# Autodesk Inventor assembly: Full payload assembly mk 2
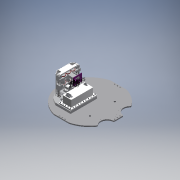
[picture p0: Inventor's stored thumbnail of the model, 180x180]
Saved by Autodesk Inventor 2017 (Build 210142000, 142)
## iProperties
Created: 2016-12-06
Part Number: Full payload assembly mk 2
Document SubType Name: Assembly
Designer: qupec
Mass: 1513.48 g
Surface Area: 2866.97 cm^2
Volume: 582.995 cm^3
Density: 2.59604 g/cm^3
Author: qupec
## Documents named in this file (42)
- C:\UMD\BPP\ROCKSAT X\STAR\CAD\Mechanical\Full payload assembly\Full payload assembly.iam
- C:\UMD\BPP\ROCKSAT X\STAR\CAD\Mechanical\Full payload assembly\Subsystems\Slide Rods\Slide rod assembly.iam
- C:\UMD\BPP\ROCKSAT X\STAR\CAD\Mechanical\Full payload assembly\Subsystems\Test Tube Rack\Test tube rack.iam
- C:\UMD\BPP\ROCKSAT X\STAR\CAD\Mechanical\Full payload assembly\Subsystems\Electronics\Electronics Stack.iam
- C:\UMD\BPP\ROCKSAT X\STAR\CAD\Mechanical\Full payload assembly\Subsystems\Video Capture\Pi Cam and Cable assembly.iam
- C:\UMD\BPP\ROCKSAT X\STAR\CAD\Mechanical\Full payload assembly\Subsystems\Electronics\Ribbon Cable Connector-02.ipt
- C:\UMD\BPP\ROCKSAT X\STAR\CAD\Mechanical\Full payload assembly\Base Plate.ipt
- C:\UMD\BPP\ROCKSAT X\STAR\CAD\Mechanical\Full payload assembly\Subsystems\Electronics\Electronics Box.ipt
- C:\UMD\BPP\ROCKSAT X\STAR\CAD\Mechanical\Full payload assembly\Subsystems\Electronics\External Sensor Board.ipt
- C:\UMD\BPP\ROCKSAT X\STAR\CAD\Mechanical\Full payload assembly\Subsystems\Electronics\9pin female connector.ipt
- C:\UMD\BPP\ROCKSAT X\STAR\CAD\Mechanical\Full payload assembly\Subsystems\Electronics\31pin female connector.ipt
- C:\UMD\BPP\ROCKSAT X\STAR\CAD\Mechanical\Full payload assembly\Subsystems\Electronics\15pin female connector.ipt
- C:\UMD\BPP\ROCKSAT X\STAR\CAD\Mechanical\Full payload assembly\Subsystems\Video Capture\LED.ipt
- C:\UMD\BPP\ROCKSAT X\STAR\CAD\Mechanical\Full payload assembly\Solar Shield.ipt
- C:\UMD\BPP\ROCKSAT X\STAR\CAD\Mechanical\Full payload assembly\BRACKET.ipt
- C:\UMD\BPP\ROCKSAT X\STAR\CAD\Mechanical\Full payload assembly\Subsystems\Shaker\ShakerAssembly.iam
- C:\UMD\BPP\ROCKSAT X\STAR\CAD\Mechanical\Full payload assembly\Subsystems\Fasteners\Num4 Narrow Split Washer.ipt
- C:\UMD\BPP\ROCKSAT X\STAR\CAD\Mechanical\Full payload assembly\Subsystems\Fasteners\4-40 .5in Socket Screw.ipt
- C:\UMD\BPP\ROCKSAT X\STAR\CAD\Mechanical\Full payload assembly\Subsystems\Fasteners\4-40 .375in Countersunk Screw.ipt
- C:\UMD\BPP\ROCKSAT X\STAR\CAD\Mechanical\Full payload assembly\Subsystems\Fasteners\Num4 Flat Washer.ipt
- C:\UMD\BPP\ROCKSAT X\STAR\CAD\Mechanical\Full payload assembly\Subsystems\Fasteners\4-40 Flex Nut.ipt
- C:\UMD\BPP\ROCKSAT X\STAR\CAD\Mechanical\Full payload assembly\Subsystems\Fasteners\4-40 .375 Socket Screw.ipt
- C:\UMD\BPP\ROCKSAT X\STAR\CAD\Mechanical\Full payload assembly\RSX Deck.ipt
- C:\UMD\BPP\ROCKSAT X\STAR\CAD\Mechanical\Full payload assembly\Subsystems\Fasteners\Num10 Belville Washer.ipt
- C:\UMD\BPP\ROCKSAT X\STAR\CAD\Mechanical\Full payload assembly\Subsystems\Fasteners\10-32 .375in Low Profile Socket Screw.ipt
- C:\UMD\BPP\ROCKSAT X\STAR\CAD\Mechanical\Full payload assembly\Subsystems\Fasteners\10-32 1.125in Countersunk Screw.ipt
- C:\UMD\BPP\ROCKSAT X\STAR\CAD\Mechanical\Full payload assembly\Subsystems\Fasteners\10-32 Flex Nut.ipt
- C:\UMD\BPP\ROCKSAT X\STAR\CAD\Mechanical\Full payload assembly\Subsystems\Fasteners\M2 Insulating Washer.ipt
- C:\UMD\BPP\ROCKSAT X\STAR\CAD\Mechanical\Full payload assembly\Subsystems\Fasteners\M2x.4mm Locknut.ipt
- C:\UMD\BPP\ROCKSAT X\STAR\CAD\Mechanical\Full payload assembly\Subsystems\Fasteners\M2x.4mm 12mm Socket Screw.ipt
- C:\UMD\BPP\ROCKSAT X\star\CAD\Mechanical\Subsystems\Full payload assembly mk 2\AIP\FEA\c3occb59c.fins
- C:\UMD\BPP\ROCKSAT X\star\CAD\Mechanical\Subsystems\Full payload assembly mk 2\AIP\FEA\c3occb5b4.fsat
- C:\UMD\BPP\ROCKSAT X\star\CAD\Mechanical\Subsystems\Full payload assembly mk 2\AIP\FEA\c3occb5b4.ftes
- C:\UMD\BPP\ROCKSAT X\star\CAD\Mechanical\Subsystems\Full payload assembly mk 2\AIP\FEA\c3occb5b4.fwiz
- C:\UMD\BPP\ROCKSAT X\star\CAD\Mechanical\Subsystems\Full payload assembly mk 2\AIP\FEA\c3occb5c0.fins
- C:\UMD\BPP\ROCKSAT X\star\CAD\Mechanical\Subsystems\Full payload assembly mk 2\AIP\FEA\c3occb5c0.fsat
- C:\UMD\BPP\ROCKSAT X\star\CAD\Mechanical\Subsystems\Full payload assembly mk 2\AIP\FEA\c3occb5c0.ftes
- C:\UMD\BPP\ROCKSAT X\star\CAD\Mechanical\Subsystems\Full payload assembly mk 2\AIP\FEA\c3occb5c0.fwiz
- C:\UMD\BPP\ROCKSAT X\star\CAD\Mechanical\Subsystems\Full payload assembly mk 2\AIP\FEA\c3occb60w.fmsh
- C:\UMD\BPP\ROCKSAT X\star\CAD\Mechanical\Subsystems\Full payload assembly mk 2\AIP\FEA\c3occb60x.fres
- C:\UMD\BPP\ROCKSAT X\star\CAD\Mechanical\Subsystems\Full payload assembly mk 2\AIP\FEA\c3occb6sg.fmsh
- C:\UMD\BPP\ROCKSAT X\star\CAD\Mechanical\Subsystems\Full payload assembly mk 2\AIP\FEA\c3occb6sh.fres
## Components (134 placed, 29 different names)
1. Slide rod assembly:1 [sub-assembly] — Mate:121, Flush:47, Mate:382, Mate:398, Mate:399, Flush:48
2. Test tube rack:1 [sub-assembly] — Mate:56, Flush:19, Flush:20, Flush:45, Mate:395, Mate:396, Mate:398, Mate:399, Mate:629, Mate:632, Mate:633, Mate:637, Mate:638
3. Pi Cam and Cable assembly:1 [sub-assembly] — Mate:56, Flush:19, Flush:20, Mate:299, Mate:300, Mate:302, Mate:303, Mate:304, Mate:593, Mate:594, Mate:595, Mate:596, Mate:597, Mate:598, Mate:599, Mate:600, Mate:606, Mate:625, Mate:626, Mate:627, Mate:628, Mate:630, Mate:631, Mate:636
4. Ribbon Cable Connector-02:1 — Mate:80, Flush:24, Flush:25
5. Electronics Stack:1 [sub-assembly] — Mate:80, Flush:24, Flush:25, Flush:41, Flush:42, Mate:397
6. Base Plate:1 — Mate:121, Mate:124, Flush:29, Flush:32, Mate:163, Flush:33, Flush:40, Flush:45, Mate:386, Mate:389, Mate:392, Mate:393, Mate:394, Mate:397, Mate:559, Mate:560, Mate:561, Mate:589, Mate:590, Mate:591, Mate:592
7. External Sensor Board:1 — Angle:1, Mate:303, Mate:304, Mate:305, Mate:306, Mate:609, Mate:610, Mate:611, Mate:612, Mate:613, Mate:614, Mate:615, Mate:616
8. 31pin female connector:1 — Flush:34, Flush:35, Mate:164
9. 15pin female connector:1 — Mate:165, Flush:43, Flush:44
10. 9pin female connector:1 — Flush:38, Flush:39, Mate:166
11. Electronics Box:1 — Mate:163, Flush:33, Flush:34, Flush:35, Mate:164, Flush:38, Flush:39, Mate:165, Mate:166, Flush:40, Flush:41, Flush:42, Flush:43, Flush:44, Mate:400, Mate:401, Mate:402, Mate:403, Mate:404, Mate:405, Mate:406, Mate:407, Mate:408, Mate:409, Mate:410, Mate:411, Mate:412, Mate:413, Mate:414, Mate:415, Mate:416, Mate:417, Mate:418, Mate:419, Mate:420, Mate:421, Mate:422, Mate:423, Mate:424, Mate:425, Mate:426, Mate:427, Mate:428, Mate:429, Mate:430, Mate:431, Mate:432, Mate:433, Mate:434, Mate:435, Mate:437, Mate:438, Mate:439, Mate:440, Mate:441, Mate:442, Mate:443, Mate:444, Mate:445, Mate:446, Mate:447, Mate:448, Mate:449, Mate:450, Mate:451, Mate:452, Mate:453, Mate:454, Mate:455, Mate:456, Mate:457, Mate:458, Mate:459, Mate:518
12. LED:1 — Mate:299, Mate:301, Mate:302, Mate:305
13. LED:2 — Mate:300, Mate:301, Mate:306
14. Solar Shield:1 — Flush:47, Mate:382, Mate:387, Mate:388, Mate:390, Mate:391, Mate:536, Mate:538, Mate:540, Mate:542, Mate:551, Mate:552, Mate:553, Mate:554, Mate:557, Mate:558, Flush:48
15. BRACKET:1 — Mate:389, Mate:390, Mate:391, Mate:519, Mate:520, Mate:521, Mate:522, Mate:527, Mate:528, Mate:529, Mate:530
16. BRACKET:2 — Mate:386, Mate:387, Mate:388, Mate:523, Mate:524, Mate:525, Mate:526, Mate:531, Mate:532, Mate:533, Mate:534
17. ShakerAssembly:1 [sub-assembly] — Mate:392, Mate:393, Mate:394, Mate:395, Mate:396
18. Num4 Narrow Split Washer:1 — Mate:411, Mate:457, Mate:645
19. Num4 Narrow Split Washer:2 — Mate:413, Mate:419, Mate:455
20. Num4 Narrow Split Washer:3 — Mate:415, Mate:450
21. Num4 Narrow Split Washer:4 — Mate:414, Mate:444
22. Num4 Narrow Split Washer:5 — Mate:412, Mate:452
23. Num4 Narrow Split Washer:6 — Mate:410, Mate:443
24. Num4 Narrow Split Washer:7 — Mate:409, Mate:453
25. Num4 Narrow Split Washer:8 — Mate:408, Mate:441
26. Num4 Narrow Split Washer:9 — Mate:420, Mate:437
27. Num4 Narrow Split Washer:10 — Mate:423, Mate:451
28. Num4 Narrow Split Washer:11 — Mate:407, Mate:445
29. Num4 Narrow Split Washer:12 — Mate:405, Mate:447
30. Num4 Narrow Split Washer:13 — Mate:428, Mate:433
31. Num4 Narrow Split Washer:14 — Mate:426, Mate:435
32. Num4 Narrow Split Washer:15 — Mate:418, Mate:430
33. Num4 Narrow Split Washer:17 — Mate:422, Mate:454
34. Num4 Narrow Split Washer:18 — Mate:417, Mate:431
35. Num4 Narrow Split Washer:19 — Mate:425, Mate:456
36. Num4 Narrow Split Washer:20 — Mate:424, Mate:439
37. Num4 Narrow Split Washer:21 — Mate:427, Mate:434
38. Num4 Narrow Split Washer:22 — Mate:429, Mate:432
39. Num4 Narrow Split Washer:23 — Mate:421, Mate:438
40. Num4 Narrow Split Washer:24 — Mate:404, Mate:440
41. Num4 Narrow Split Washer:25 — Mate:401, Mate:442
42. Num4 Narrow Split Washer:26 — Mate:400, Mate:416, Mate:449
43. Num4 Narrow Split Washer:27 — Mate:402, Mate:406, Mate:446
44. Num4 Narrow Split Washer:28 — Mate:403, Mate:448
45. Num4 Narrow Split Washer:29 — Mate:458, Mate:459
46. 4-40 .5in Socket Screw:1
47. 4-40 .5in Socket Screw:2
48. 4-40 .5in Socket Screw:3
49. 4-40 .5in Socket Screw:4
50. 4-40 .5in Socket Screw:5
51. 4-40 .5in Socket Screw:6
52. 4-40 .5in Socket Screw:7
53. 4-40 .5in Socket Screw:8
54. 4-40 .5in Socket Screw:9
55. 4-40 .5in Socket Screw:10
56. 4-40 .5in Socket Screw:11
57. 4-40 .5in Socket Screw:12
58. 4-40 .5in Socket Screw:13
59. 4-40 .5in Socket Screw:14
60. 4-40 .5in Socket Screw:15 — Mate:518
61. 4-40 .5in Socket Screw:16
62. 4-40 .5in Socket Screw:17 — Mate:645
63. 4-40 .5in Socket Screw:18
64. 4-40 .5in Socket Screw:19
65. 4-40 .5in Socket Screw:20
66. 4-40 .5in Socket Screw:21
67. 4-40 .5in Socket Screw:22
68. 4-40 .5in Socket Screw:23
69. 4-40 .5in Socket Screw:24
70. 4-40 .5in Socket Screw:25
71. 4-40 .5in Socket Screw:26
72. 4-40 .5in Socket Screw:27
73. 4-40 .5in Socket Screw:28
74. 4-40 .375in Countersunk Screw:1 — Mate:520, Mate:521
75. 4-40 .375in Countersunk Screw:2 — Mate:519, Mate:522
76. 4-40 .375in Countersunk Screw:3 — Mate:523, Mate:526
77. 4-40 .375in Countersunk Screw:4 — Mate:524, Mate:525
78. 4-40 .375in Countersunk Screw:5 — Mate:531, Mate:534, Mate:537, Mate:546
79. 4-40 .375in Countersunk Screw:6 — Mate:528, Mate:529, Mate:541, Mate:550
80. 4-40 .375in Countersunk Screw:7 — Mate:532, Mate:533, Mate:535, Mate:543
81. 4-40 .375in Countersunk Screw:8 — Mate:527, Mate:530, Mate:539, Mate:548
82. Num4 Flat Washer:1 — Mate:539, Mate:540, Mate:547
83. Num4 Flat Washer:2 — Mate:537, Mate:538, Mate:545
84. Num4 Flat Washer:3 — Mate:535, Mate:536, Mate:544
85. Num4 Flat Washer:4 — Mate:541, Mate:542, Mate:549
86. 4-40 Flex Nut:1 — Mate:549, Mate:550
87. 4-40 Flex Nut:2 — Mate:545, Mate:546
88. 4-40 Flex Nut:3 — Mate:547, Mate:548
89. 4-40 Flex Nut:4 — Mate:543, Mate:544
90. Num4 Narrow Split Washer:30 — Mate:551, Mate:552, Mate:556
91. Num4 Narrow Split Washer:31 — Mate:553, Mate:554, Mate:555
92. 4-40 .375 Socket Screw:1 — Mate:555, Mate:558
93. 4-40 .375 Socket Screw:2 — Mate:556, Mate:557
94. RSX Deck:1 — Mate:559, Mate:560, Mate:561, Mate:562, Mate:563, Mate:565, Mate:566, Mate:567, Mate:568, Mate:569, Mate:570, Mate:571, Mate:575, Mate:577, Mate:578, Mate:579, Mate:580, Mate:581, Mate:582, Mate:583, Mate:584
95. Num10 Belville Washer:1 — Mate:562, Mate:563, Mate:574
96. Num10 Belville Washer:3 — Mate:565, Mate:566, Mate:573
97. Num10 Belville Washer:4 — Mate:567, Mate:568, Mate:572
98. 10-32 .375in Low Profile Socket Screw:1 — Mate:569, Mate:574
99. 10-32 .375in Low Profile Socket Screw:2 — Mate:570, Mate:573
100. 10-32 .375in Low Profile Socket Screw:3 — Mate:571, Mate:572
101. 10-32 1.125in Countersunk Screw:1 — Mate:575, Mate:581, Mate:582, Mate:585
102. 10-32 1.125in Countersunk Screw:2 — Mate:577, Mate:584, Mate:587
103. 10-32 1.125in Countersunk Screw:3 — Mate:579, Mate:580, Mate:586
104. 10-32 1.125in Countersunk Screw:4 — Mate:578, Mate:583, Mate:588
105. 10-32 Flex Nut:1 — Mate:586, Mate:589
106. 10-32 Flex Nut:2 — Mate:587, Mate:592
107. 10-32 Flex Nut:3 — Mate:588, Mate:591
108. 10-32 Flex Nut:4 — Mate:585, Mate:590
109. M2 Insulating Washer:1 — Mate:593, Mate:594, Mate:603, Mate:604
110. M2 Insulating Washer:2 — Mate:599, Mate:600, Mate:607, Mate:608
111. M2 Insulating Washer:3 — Mate:597, Mate:598, Mate:605
112. M2 Insulating Washer:4 — Mate:595, Mate:596, Mate:601, Mate:602
113. M2x.4mm Locknut:1 — Mate:601, Mate:602
114. M2x.4mm Locknut:2 — Mate:603, Mate:604
115. M2x.4mm Locknut:3 — Mate:607, Mate:608
116. M2x.4mm Locknut:4 — Mate:605, Mate:606
117. M2x.4mm 12mm Socket Screw:1 — Mate:610, Mate:619, Mate:623
118. M2x.4mm 12mm Socket Screw:2 — Mate:609, Mate:618, Mate:621
119. M2x.4mm 12mm Socket Screw:3 — Mate:611, Mate:617, Mate:622
120. M2x.4mm 12mm Socket Screw:4 — Mate:612, Mate:620, Mate:624
121. M2 Insulating Washer:5 — Mate:616, Mate:617
122. M2 Insulating Washer:6 — Mate:614, Mate:619
123. M2 Insulating Washer:7 — Mate:613, Mate:620, Mate:624
124. M2 Insulating Washer:8 — Mate:615, Mate:618, Mate:621, Mate:622, Mate:623
125. Num4 Flat Washer:5 — Mate:625, Mate:630, Mate:634, Mate:635
126. Num4 Flat Washer:6 — Mate:627, Mate:629
127. Num4 Flat Washer:7 — Mate:626, Mate:628
128. 4-40 .5in Socket Screw:29 — Mate:631, Mate:636, Mate:639, Mate:644
129. 4-40 .5in Socket Screw:30 — Mate:632, Mate:634, Mate:640, Mate:643
130. 4-40 .5in Socket Screw:31 — Mate:633, Mate:635
131. Num4 Flat Washer:8 — Mate:637, Mate:640, Mate:642
132. Num4 Flat Washer:9 — Mate:638, Mate:639, Mate:641
133. 4-40 Flex Nut:5 — Mate:642, Mate:643
134. 4-40 Flex Nut:6 — Mate:641, Mate:644
## Relationships (291: Mate 271, Flush 19, Angle 1)
- Mate:56: Test tube rack:1 ↔ Pi Cam and Cable assembly:1
- Flush:19: Test tube rack:1 ↔ Pi Cam and Cable assembly:1
- Flush:20: Test tube rack:1 ↔ Pi Cam and Cable assembly:1
- Mate:80: Ribbon Cable Connector-02:1 ↔ Electronics Stack:1
- Flush:24 (-7 mm): Ribbon Cable Connector-02:1 ↔ Electronics Stack:1
- Flush:25: Ribbon Cable Connector-02:1 ↔ Electronics Stack:1
- Mate:121: Slide rod assembly:1 ↔ Base Plate:1
- Mate:124: Base Plate:1
- Flush:29: Base Plate:1
- Flush:32: Base Plate:1
- Angle:1 (0 deg): External Sensor Board:1
- Mate:163: Base Plate:1 ↔ Electronics Box:1
- Flush:33: Base Plate:1 ↔ Electronics Box:1
- Flush:34 (12.7 mm): 31pin female connector:1 ↔ Electronics Box:1
- Flush:35 (6.35 mm): 31pin female connector:1 ↔ Electronics Box:1
- Mate:164: 31pin female connector:1 ↔ Electronics Box:1
- Flush:38 (6.35 mm): 9pin female connector:1 ↔ Electronics Box:1
- Flush:39 (-6.35 mm): 9pin female connector:1 ↔ Electronics Box:1
- Mate:165: 15pin female connector:1 ↔ Electronics Box:1
- Mate:166: 9pin female connector:1 ↔ Electronics Box:1
- Flush:40: Base Plate:1 ↔ Electronics Box:1
- Flush:41 (3.175 mm): Electronics Stack:1 ↔ Electronics Box:1
- Flush:42: Electronics Stack:1 ↔ Electronics Box:1
- Flush:43 (3.81 mm): 15pin female connector:1 ↔ Electronics Box:1
- Flush:44 (12.7 mm): 15pin female connector:1 ↔ Electronics Box:1
- Mate:299: Pi Cam and Cable assembly:1 ↔ LED:1
- Mate:300: Pi Cam and Cable assembly:1 ↔ LED:2
- Mate:301: LED:1 ↔ LED:2
- Mate:302: Pi Cam and Cable assembly:1 ↔ LED:1
- Mate:303: Pi Cam and Cable assembly:1 ↔ External Sensor Board:1
- Mate:304: Pi Cam and Cable assembly:1 ↔ External Sensor Board:1
- Mate:305: External Sensor Board:1 ↔ LED:1
- Mate:306: External Sensor Board:1 ↔ LED:2
- Flush:45: Test tube rack:1 ↔ Base Plate:1
- Flush:47: Slide rod assembly:1 ↔ Solar Shield:1
- Mate:382: Slide rod assembly:1 ↔ Solar Shield:1
- Mate:386: Base Plate:1 ↔ BRACKET:2
- Mate:387: Solar Shield:1 ↔ BRACKET:2
- Mate:388 (3.175 mm): Solar Shield:1 ↔ BRACKET:2
- Mate:389: Base Plate:1 ↔ BRACKET:1
- Mate:390: Solar Shield:1 ↔ BRACKET:1
- Mate:391 (3.175 mm): Solar Shield:1 ↔ BRACKET:1
- Mate:392: Base Plate:1 ↔ ShakerAssembly:1
- Mate:393: Base Plate:1 ↔ ShakerAssembly:1
- Mate:394: Base Plate:1 ↔ ShakerAssembly:1
- Mate:395: Test tube rack:1 ↔ ShakerAssembly:1
- Mate:396: Test tube rack:1 ↔ ShakerAssembly:1
- Mate:397: Electronics Stack:1 ↔ Base Plate:1
- Mate:398: Slide rod assembly:1 ↔ Test tube rack:1
- Mate:399: Slide rod assembly:1 ↔ Test tube rack:1
- Mate:400: Electronics Box:1 ↔ Num4 Narrow Split Washer:26
- Mate:401: Electronics Box:1 ↔ Num4 Narrow Split Washer:25
- Mate:402: Electronics Box:1 ↔ Num4 Narrow Split Washer:27
- Mate:403: Electronics Box:1 ↔ Num4 Narrow Split Washer:28
- Mate:404: Electronics Box:1 ↔ Num4 Narrow Split Washer:24
- Mate:405: Electronics Box:1 ↔ Num4 Narrow Split Washer:12
- Mate:406: Electronics Box:1 ↔ Num4 Narrow Split Washer:27
- Mate:407: Electronics Box:1 ↔ Num4 Narrow Split Washer:11
- Mate:408: Electronics Box:1 ↔ Num4 Narrow Split Washer:8
- Mate:409: Electronics Box:1 ↔ Num4 Narrow Split Washer:7
- Mate:410: Electronics Box:1 ↔ Num4 Narrow Split Washer:6
- Mate:411: Electronics Box:1 ↔ Num4 Narrow Split Washer:1
- Mate:412: Electronics Box:1 ↔ Num4 Narrow Split Washer:5
- Mate:413: Electronics Box:1 ↔ Num4 Narrow Split Washer:2
- Mate:414: Electronics Box:1 ↔ Num4 Narrow Split Washer:4
- Mate:415: Electronics Box:1 ↔ Num4 Narrow Split Washer:3
- Mate:416: Electronics Box:1 ↔ Num4 Narrow Split Washer:26
- Mate:417: Electronics Box:1 ↔ Num4 Narrow Split Washer:18
- Mate:418: Electronics Box:1 ↔ Num4 Narrow Split Washer:15
- Mate:419: Electronics Box:1 ↔ Num4 Narrow Split Washer:2
- Mate:420: Electronics Box:1 ↔ Num4 Narrow Split Washer:9
- Mate:421: Electronics Box:1 ↔ Num4 Narrow Split Washer:23
- Mate:422: Electronics Box:1 ↔ Num4 Narrow Split Washer:17
- Mate:423: Electronics Box:1 ↔ Num4 Narrow Split Washer:10
- Mate:424: Electronics Box:1 ↔ Num4 Narrow Split Washer:20
- Mate:425: Electronics Box:1 ↔ Num4 Narrow Split Washer:19
- Mate:426: Electronics Box:1 ↔ Num4 Narrow Split Washer:14
- Mate:427: Electronics Box:1 ↔ Num4 Narrow Split Washer:21
- Mate:428: Electronics Box:1 ↔ Num4 Narrow Split Washer:13
- Mate:429: Electronics Box:1 ↔ Num4 Narrow Split Washer:22
- Mate:430: Electronics Box:1 ↔ Num4 Narrow Split Washer:15
- Mate:431: Electronics Box:1 ↔ Num4 Narrow Split Washer:18
- Mate:432: Electronics Box:1 ↔ Num4 Narrow Split Washer:22
- Mate:433: Electronics Box:1 ↔ Num4 Narrow Split Washer:13
- Mate:434: Electronics Box:1 ↔ Num4 Narrow Split Washer:21
- Mate:435: Electronics Box:1 ↔ Num4 Narrow Split Washer:14
- Mate:437: Electronics Box:1 ↔ Num4 Narrow Split Washer:9
- Mate:438: Electronics Box:1 ↔ Num4 Narrow Split Washer:23
- Mate:439: Electronics Box:1 ↔ Num4 Narrow Split Washer:20
- Mate:440: Electronics Box:1 ↔ Num4 Narrow Split Washer:24
- Mate:441: Electronics Box:1 ↔ Num4 Narrow Split Washer:8
- Mate:442: Electronics Box:1 ↔ Num4 Narrow Split Washer:25
- Mate:443: Electronics Box:1 ↔ Num4 Narrow Split Washer:6
- Mate:444: Electronics Box:1 ↔ Num4 Narrow Split Washer:4
- Mate:445: Electronics Box:1 ↔ Num4 Narrow Split Washer:11
- Mate:446: Electronics Box:1 ↔ Num4 Narrow Split Washer:27
- Mate:447: Electronics Box:1 ↔ Num4 Narrow Split Washer:12
- Mate:448: Electronics Box:1 ↔ Num4 Narrow Split Washer:28
- Mate:449: Electronics Box:1 ↔ Num4 Narrow Split Washer:26
- Mate:450: Electronics Box:1 ↔ Num4 Narrow Split Washer:3
- Mate:451: Electronics Box:1 ↔ Num4 Narrow Split Washer:10
- Mate:452: Electronics Box:1 ↔ Num4 Narrow Split Washer:5
- Mate:453: Electronics Box:1 ↔ Num4 Narrow Split Washer:7
- Mate:454: Electronics Box:1 ↔ Num4 Narrow Split Washer:17
- Mate:455: Electronics Box:1 ↔ Num4 Narrow Split Washer:2
- Mate:456: Electronics Box:1 ↔ Num4 Narrow Split Washer:19
- Mate:457: Electronics Box:1 ↔ Num4 Narrow Split Washer:1
- Mate:458: Electronics Box:1 ↔ Num4 Narrow Split Washer:29
- Mate:459: Electronics Box:1 ↔ Num4 Narrow Split Washer:29
- [Mate]: Num4 Narrow Split Washer:29 ↔ 4-40 .5in Socket Screw:13
- [Mate]: Num4 Narrow Split Washer:4 ↔ 4-40 .5in Socket Screw:5
- [Mate]: Num4 Narrow Split Washer:20 ↔ 4-40 .5in Socket Screw:4
- [Mate]: Num4 Narrow Split Washer:9 ↔ 4-40 .5in Socket Screw:26
- [Mate]: Num4 Narrow Split Washer:14 ↔ 4-40 .5in Socket Screw:1
- [Mate]: Num4 Narrow Split Washer:21 ↔ 4-40 .5in Socket Screw:11
- [Mate]: Num4 Narrow Split Washer:13 ↔ 4-40 .5in Socket Screw:2
- [Mate]: Num4 Narrow Split Washer:22 ↔ 4-40 .5in Socket Screw:23
- [Mate]: Num4 Narrow Split Washer:18 ↔ 4-40 .5in Socket Screw:22
- [Mate]: Num4 Narrow Split Washer:15 ↔ 4-40 .5in Socket Screw:28
- [Mate]: Num4 Narrow Split Washer:24 ↔ 4-40 .5in Socket Screw:16
- [Mate]: Num4 Narrow Split Washer:8 ↔ 4-40 .5in Socket Screw:14
- [Mate]: Num4 Narrow Split Washer:25 ↔ 4-40 .5in Socket Screw:15
- [Mate]: Num4 Narrow Split Washer:6 ↔ 4-40 .5in Socket Screw:24
- [Mate]: Num4 Narrow Split Washer:11 ↔ 4-40 .5in Socket Screw:9
- [Mate]: Num4 Narrow Split Washer:27 ↔ 4-40 .5in Socket Screw:21
- [Mate]: Num4 Narrow Split Washer:12 ↔ 4-40 .5in Socket Screw:18
- [Mate]: Num4 Narrow Split Washer:28 ↔ 4-40 .5in Socket Screw:19
- [Mate]: Num4 Narrow Split Washer:26 ↔ 4-40 .5in Socket Screw:20
- [Mate]: Num4 Narrow Split Washer:3 ↔ 4-40 .5in Socket Screw:25
- [Mate]: Num4 Narrow Split Washer:10 ↔ 4-40 .5in Socket Screw:8
- [Mate]: Num4 Narrow Split Washer:5 ↔ 4-40 .5in Socket Screw:10
- [Mate]: Num4 Narrow Split Washer:7 ↔ 4-40 .5in Socket Screw:7
- [Mate]: Num4 Narrow Split Washer:17 ↔ 4-40 .5in Socket Screw:3
- [Mate]: Num4 Narrow Split Washer:2 ↔ 4-40 .5in Socket Screw:12
- [Mate]: Num4 Narrow Split Washer:19 ↔ 4-40 .5in Socket Screw:6
- [Mate]: Num4 Narrow Split Washer:1 ↔ 4-40 .5in Socket Screw:17
- [Mate]: Electronics Box:1 ↔ 4-40 .5in Socket Screw:24
- [Mate]: Electronics Box:1 ↔ 4-40 .5in Socket Screw:14
- [Mate]: Electronics Box:1 ↔ 4-40 .5in Socket Screw:16
- [Mate]: Electronics Box:1 ↔ 4-40 .5in Socket Screw:28
- [Mate]: Electronics Box:1 ↔ 4-40 .5in Socket Screw:22
- [Mate]: Electronics Box:1 ↔ 4-40 .5in Socket Screw:23
- [Mate]: Electronics Box:1 ↔ 4-40 .5in Socket Screw:2
- [Mate]: Electronics Box:1 ↔ 4-40 .5in Socket Screw:11
- [Mate]: Num4 Narrow Split Washer:14 ↔ 4-40 .5in Socket Screw:1
- [Mate]: Num4 Narrow Split Washer:9 ↔ 4-40 .5in Socket Screw:26
- [Mate]: Num4 Narrow Split Washer:23 ↔ 4-40 .5in Socket Screw:27
- [Mate]: Electronics Box:1 ↔ 4-40 .5in Socket Screw:27
- [Mate]: Num4 Narrow Split Washer:20 ↔ 4-40 .5in Socket Screw:4
- [Mate]: Num4 Narrow Split Washer:4 ↔ 4-40 .5in Socket Screw:5
- [Mate]: Num4 Narrow Split Washer:29 ↔ 4-40 .5in Socket Screw:13
- [Mate]: Num4 Narrow Split Washer:11 ↔ 4-40 .5in Socket Screw:9
- [Mate]: Num4 Narrow Split Washer:27 ↔ 4-40 .5in Socket Screw:21
- [Mate]: Num4 Narrow Split Washer:12 ↔ 4-40 .5in Socket Screw:18
- [Mate]: Num4 Narrow Split Washer:28 ↔ 4-40 .5in Socket Screw:19
- [Mate]: Num4 Narrow Split Washer:26 ↔ 4-40 .5in Socket Screw:20
- [Mate]: Num4 Narrow Split Washer:3 ↔ 4-40 .5in Socket Screw:25
- [Mate]: Electronics Box:1 ↔ 4-40 .5in Socket Screw:8
- [Mate]: Electronics Box:1 ↔ 4-40 .5in Socket Screw:10
- [Mate]: Num4 Narrow Split Washer:7 ↔ 4-40 .5in Socket Screw:7
- [Mate]: Num4 Narrow Split Washer:17 ↔ 4-40 .5in Socket Screw:3
- [Mate]: Num4 Narrow Split Washer:2 ↔ 4-40 .5in Socket Screw:12
- [Mate]: Num4 Narrow Split Washer:19 ↔ 4-40 .5in Socket Screw:6
- [Mate]: Num4 Narrow Split Washer:29 ↔ 4-40 .5in Socket Screw:13
- Mate:518: Electronics Box:1 ↔ 4-40 .5in Socket Screw:15
- Mate:519: BRACKET:1 ↔ 4-40 .375in Countersunk Screw:2
- Mate:520: BRACKET:1 ↔ 4-40 .375in Countersunk Screw:1
- Mate:521: BRACKET:1 ↔ 4-40 .375in Countersunk Screw:1
- Mate:522: BRACKET:1 ↔ 4-40 .375in Countersunk Screw:2
- Mate:523: BRACKET:2 ↔ 4-40 .375in Countersunk Screw:3
- Mate:524: BRACKET:2 ↔ 4-40 .375in Countersunk Screw:4
- Mate:525: BRACKET:2 ↔ 4-40 .375in Countersunk Screw:4
- Mate:526: BRACKET:2 ↔ 4-40 .375in Countersunk Screw:3
- Mate:527: BRACKET:1 ↔ 4-40 .375in Countersunk Screw:8
- Mate:528: BRACKET:1 ↔ 4-40 .375in Countersunk Screw:6
- Mate:529: BRACKET:1 ↔ 4-40 .375in Countersunk Screw:6
- Mate:530: BRACKET:1 ↔ 4-40 .375in Countersunk Screw:8
- Mate:531: BRACKET:2 ↔ 4-40 .375in Countersunk Screw:5
- Mate:532: BRACKET:2 ↔ 4-40 .375in Countersunk Screw:7
- Mate:533: BRACKET:2 ↔ 4-40 .375in Countersunk Screw:7
- Mate:534: BRACKET:2 ↔ 4-40 .375in Countersunk Screw:5
- Mate:535: 4-40 .375in Countersunk Screw:7 ↔ Num4 Flat Washer:3
- Mate:536: Solar Shield:1 ↔ Num4 Flat Washer:3
- Mate:537: 4-40 .375in Countersunk Screw:5 ↔ Num4 Flat Washer:2
- Mate:538: Solar Shield:1 ↔ Num4 Flat Washer:2
- Mate:539: 4-40 .375in Countersunk Screw:8 ↔ Num4 Flat Washer:1
- Mate:540: Solar Shield:1 ↔ Num4 Flat Washer:1
- Mate:541: 4-40 .375in Countersunk Screw:6 ↔ Num4 Flat Washer:4
- Mate:542: Solar Shield:1 ↔ Num4 Flat Washer:4
- Mate:543: 4-40 .375in Countersunk Screw:7 ↔ 4-40 Flex Nut:4
- Mate:544: Num4 Flat Washer:3 ↔ 4-40 Flex Nut:4
- Mate:545: Num4 Flat Washer:2 ↔ 4-40 Flex Nut:2
- Mate:546: 4-40 .375in Countersunk Screw:5 ↔ 4-40 Flex Nut:2
- Mate:547: Num4 Flat Washer:1 ↔ 4-40 Flex Nut:3
- Mate:548: 4-40 .375in Countersunk Screw:8 ↔ 4-40 Flex Nut:3
- Mate:549: Num4 Flat Washer:4 ↔ 4-40 Flex Nut:1
- Mate:550: 4-40 .375in Countersunk Screw:6 ↔ 4-40 Flex Nut:1
- Mate:551: Solar Shield:1 ↔ Num4 Narrow Split Washer:30
- Mate:552: Solar Shield:1 ↔ Num4 Narrow Split Washer:30
- Mate:553: Solar Shield:1 ↔ Num4 Narrow Split Washer:31
- Mate:554: Solar Shield:1 ↔ Num4 Narrow Split Washer:31
- Mate:555: Num4 Narrow Split Washer:31 ↔ 4-40 .375 Socket Screw:1
- Mate:556: Num4 Narrow Split Washer:30 ↔ 4-40 .375 Socket Screw:2
- Mate:557: Solar Shield:1 ↔ 4-40 .375 Socket Screw:2
- Mate:558: Solar Shield:1 ↔ 4-40 .375 Socket Screw:1
- Flush:48: Slide rod assembly:1 ↔ Solar Shield:1
- Mate:559: Base Plate:1 ↔ RSX Deck:1
- Mate:560: Base Plate:1 ↔ RSX Deck:1
- Mate:561: Base Plate:1 ↔ RSX Deck:1
- Mate:562: RSX Deck:1 ↔ Num10 Belville Washer:1
- Mate:563: RSX Deck:1 ↔ Num10 Belville Washer:1
- Mate:565: RSX Deck:1 ↔ Num10 Belville Washer:3
- Mate:566: RSX Deck:1 ↔ Num10 Belville Washer:3
- Mate:567: RSX Deck:1 ↔ Num10 Belville Washer:4
- Mate:568: RSX Deck:1 ↔ Num10 Belville Washer:4
- Mate:569: RSX Deck:1 ↔ 10-32 .375in Low Profile Socket Screw:1
- Mate:570: RSX Deck:1 ↔ 10-32 .375in Low Profile Socket Screw:2
- Mate:571: RSX Deck:1 ↔ 10-32 .375in Low Profile Socket Screw:3
- Mate:572: Num10 Belville Washer:4 ↔ 10-32 .375in Low Profile Socket Screw:3
- Mate:573: Num10 Belville Washer:3 ↔ 10-32 .375in Low Profile Socket Screw:2
- Mate:574: Num10 Belville Washer:1 ↔ 10-32 .375in Low Profile Socket Screw:1
- Mate:575: RSX Deck:1 ↔ 10-32 1.125in Countersunk Screw:1
- Mate:577: RSX Deck:1 ↔ 10-32 1.125in Countersunk Screw:2
- Mate:578: RSX Deck:1 ↔ 10-32 1.125in Countersunk Screw:4
- Mate:579: RSX Deck:1 ↔ 10-32 1.125in Countersunk Screw:3
- Mate:580: RSX Deck:1 ↔ 10-32 1.125in Countersunk Screw:3
- Mate:581: RSX Deck:1 ↔ 10-32 1.125in Countersunk Screw:1
- Mate:582: RSX Deck:1 ↔ 10-32 1.125in Countersunk Screw:1
- Mate:583: RSX Deck:1 ↔ 10-32 1.125in Countersunk Screw:4
- Mate:584: RSX Deck:1 ↔ 10-32 1.125in Countersunk Screw:2
- Mate:585: 10-32 1.125in Countersunk Screw:1 ↔ 10-32 Flex Nut:4
- Mate:586: 10-32 1.125in Countersunk Screw:3 ↔ 10-32 Flex Nut:1
- Mate:587: 10-32 1.125in Countersunk Screw:2 ↔ 10-32 Flex Nut:2
- Mate:588: 10-32 1.125in Countersunk Screw:4 ↔ 10-32 Flex Nut:3
- Mate:589: Base Plate:1 ↔ 10-32 Flex Nut:1
- Mate:590: Base Plate:1 ↔ 10-32 Flex Nut:4
- Mate:591: Base Plate:1 ↔ 10-32 Flex Nut:3
- Mate:592: Base Plate:1 ↔ 10-32 Flex Nut:2
- Mate:593: Pi Cam and Cable assembly:1 ↔ M2 Insulating Washer:1
- Mate:594: Pi Cam and Cable assembly:1 ↔ M2 Insulating Washer:1
- Mate:595: Pi Cam and Cable assembly:1 ↔ M2 Insulating Washer:4
- Mate:596: Pi Cam and Cable assembly:1 ↔ M2 Insulating Washer:4
- Mate:597: Pi Cam and Cable assembly:1 ↔ M2 Insulating Washer:3
- Mate:598: Pi Cam and Cable assembly:1 ↔ M2 Insulating Washer:3
- Mate:599: Pi Cam and Cable assembly:1 ↔ M2 Insulating Washer:2
- Mate:600: Pi Cam and Cable assembly:1 ↔ M2 Insulating Washer:2
- Mate:601: M2 Insulating Washer:4 ↔ M2x.4mm Locknut:1
- Mate:602: M2 Insulating Washer:4 ↔ M2x.4mm Locknut:1
- Mate:603: M2 Insulating Washer:1 ↔ M2x.4mm Locknut:2
- Mate:604: M2 Insulating Washer:1 ↔ M2x.4mm Locknut:2
- Mate:605: M2 Insulating Washer:3 ↔ M2x.4mm Locknut:4
- Mate:606: Pi Cam and Cable assembly:1 ↔ M2x.4mm Locknut:4
- Mate:607: M2 Insulating Washer:2 ↔ M2x.4mm Locknut:3
- Mate:608: M2 Insulating Washer:2 ↔ M2x.4mm Locknut:3
- Mate:609: External Sensor Board:1 ↔ M2x.4mm 12mm Socket Screw:2
- Mate:610: External Sensor Board:1 ↔ M2x.4mm 12mm Socket Screw:1
- Mate:611: External Sensor Board:1 ↔ M2x.4mm 12mm Socket Screw:3
- Mate:612: External Sensor Board:1 ↔ M2x.4mm 12mm Socket Screw:4
- Mate:613: External Sensor Board:1 ↔ M2 Insulating Washer:7
- Mate:614: External Sensor Board:1 ↔ M2 Insulating Washer:6
- Mate:615: External Sensor Board:1 ↔ M2 Insulating Washer:8
- Mate:616: External Sensor Board:1 ↔ M2 Insulating Washer:5
- Mate:617: M2x.4mm 12mm Socket Screw:3 ↔ M2 Insulating Washer:5
- Mate:618: M2x.4mm 12mm Socket Screw:2 ↔ M2 Insulating Washer:8
- Mate:619: M2x.4mm 12mm Socket Screw:1 ↔ M2 Insulating Washer:6
- Mate:620: M2x.4mm 12mm Socket Screw:4 ↔ M2 Insulating Washer:7
- Mate:621: M2x.4mm 12mm Socket Screw:2 ↔ M2 Insulating Washer:8
- Mate:622: M2x.4mm 12mm Socket Screw:3 ↔ M2 Insulating Washer:8
- Mate:623: M2x.4mm 12mm Socket Screw:1 ↔ M2 Insulating Washer:8
- Mate:624: M2x.4mm 12mm Socket Screw:4 ↔ M2 Insulating Washer:7
- Mate:625: Pi Cam and Cable assembly:1 ↔ Num4 Flat Washer:5
- Mate:626: Pi Cam and Cable assembly:1 ↔ Num4 Flat Washer:7
- Mate:627: Pi Cam and Cable assembly:1 ↔ Num4 Flat Washer:6
- Mate:628: Pi Cam and Cable assembly:1 ↔ Num4 Flat Washer:7
- Mate:629: Test tube rack:1 ↔ Num4 Flat Washer:6
- Mate:630: Pi Cam and Cable assembly:1 ↔ Num4 Flat Washer:5
- Mate:631: Pi Cam and Cable assembly:1 ↔ 4-40 .5in Socket Screw:29
- Mate:632: Test tube rack:1 ↔ 4-40 .5in Socket Screw:30
- Mate:633: Test tube rack:1 ↔ 4-40 .5in Socket Screw:31
- Mate:634: Num4 Flat Washer:5 ↔ 4-40 .5in Socket Screw:30
- Mate:635: Num4 Flat Washer:5 ↔ 4-40 .5in Socket Screw:31
- Mate:636: Pi Cam and Cable assembly:1 ↔ 4-40 .5in Socket Screw:29
- Mate:637: Test tube rack:1 ↔ Num4 Flat Washer:8
- Mate:638: Test tube rack:1 ↔ Num4 Flat Washer:9
- Mate:639: 4-40 .5in Socket Screw:29 ↔ Num4 Flat Washer:9
- Mate:640: 4-40 .5in Socket Screw:30 ↔ Num4 Flat Washer:8
- Mate:641: Num4 Flat Washer:9 ↔ 4-40 Flex Nut:6
- Mate:642: Num4 Flat Washer:8 ↔ 4-40 Flex Nut:5
- Mate:643: 4-40 .5in Socket Screw:30 ↔ 4-40 Flex Nut:5
- Mate:644: 4-40 .5in Socket Screw:29 ↔ 4-40 Flex Nut:6
- Mate:645: Num4 Narrow Split Washer:1 ↔ 4-40 .5in Socket Screw:17
## Named parameters: sa_3 = 0, sa_4 = 29260.8, sa_5 = 0, sa_6 = 6894.76
note: some values were not read from the file. Shown as the stored number, unit unknown: "sa_3", "sa_4", "sa_5", "sa_6".
